# Autodesk Inventor assembly: Assembly wiel
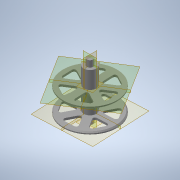
[picture p0: Inventor's stored thumbnail of the model, 180x180]
Saved by Autodesk Inventor 2021 (Build 250183000, 183)
## iProperties
Manager: PJ / DCS
Company: Emmaüs Bovenbouw Aalter
Created: 2021-01-10
Part Number: Assembly wiel
Catalog Web Link: http://emmausbovenbouw.op-weg.be/
Vendor: Emmaüs Bovenbouw Aalter
Document SubType Name: Assembly
Designer: Antho
Engineer: Declercq St.
Authority: Declercq St.
Title: Algemene Projecttitel
Author: Antho
## Documents named in this file (5)
- D:\Inventor\GIP 6EM\Assembly\Assembly wiel.iam
- D:\Inventor\GIP 6EM\Wielen\Hoes.ipt
- D:\Inventor\GIP 6EM\Wielen\Stang.ipt
- D:\Inventor\GIP 6EM\Wielen\Wiel hout.ipt
- D:\Inventor\GIP 6EM\Wielen\Kleine Hoes.ipt
## Components (5 placed, 4 different names)
1. Hoes:1 — Mate:5, Mate:6
2. Stang:1 — Mate:1, Mate:2, Mate:3, Mate:4, Mate:5, Mate:7, Mate:9, Mate:10
3. Wiel hout:1 — Mate:3, Mate:4, Mate:6, Mate:9
4. Wiel hout:2 — Mate:1, Mate:2, Mate:8, Mate:10
5. Kleine Hoes:1 — Mate:7, Mate:8
## Relationships (10: Mate 10)
- Mate:1: Stang:1 ↔ Wiel hout:2
- Mate:2: Stang:1 ↔ Wiel hout:2
- Mate:3: Stang:1 ↔ Wiel hout:1
- Mate:4: Stang:1 ↔ Wiel hout:1
- Mate:5: Hoes:1 ↔ Stang:1
- Mate:6: Hoes:1 ↔ Wiel hout:1
- Mate:7: Stang:1 ↔ Kleine Hoes:1
- Mate:8: Wiel hout:2 ↔ Kleine Hoes:1
- Mate:9: Stang:1 ↔ Wiel hout:1
- Mate:10: Stang:1 ↔ Wiel hout:2
